# Autodesk Inventor assembly: ModuloCocina_4
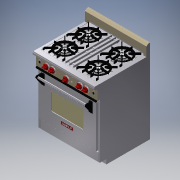
[picture p0: Inventor's stored thumbnail of the model, 180x180]
Saved by Autodesk Inventor 2016 (Build 200138000, 138)
## iProperties
Created: 2015-11-24
Part Number: ModuloCocina_4
Material: Genérico
Document SubType Name: Assembly
Designer: eolun
Author: eolun
## Documents named in this file (2)
- D:\Documents\Carrera\11.Semeste_II_2015\Computacion_grafica\Proyecto\COCINA_FINAL\Cocina\ModuloCocina_4.iam
- D:\Documents\Carrera\11.Semeste_II_2015\Computacion_grafica\Proyecto\COCINA_FINAL\Cocina\estufa_4.ipt
## Components (1 placed, 1 different names)
1. estufa_4:1 — Mate:1
## Relationships (1: Mate 1)
- Mate:1: estufa_4:1
